# Autodesk Inventor assembly: HatpHexa
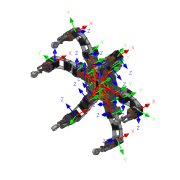
[picture p0: Inventor's stored thumbnail of the model, 180x180]
Saved by Autodesk Inventor 2019.4 (Build 234330000, 330)
## iProperties
Created: 2018-12-18
Part Number: HatpHexa
Material: 一般
Document SubType Name: Assembly
Designer: y6tada
Author: y6tada
## Documents named in this file (5)
- C:\Workspace\HaptHexa\Hardware\Inventor\HatpHexa.iam
- C:\Workspace\HaptHexa\Hardware\Inventor\Thorax\_Thorax.iam
- C:\Workspace\HaptHexa\Hardware\Inventor\Coxa\_Coxa.iam
- C:\Workspace\HaptHexa\Hardware\Inventor\Femur\_Femur.iam
- C:\Workspace\HaptHexa\Hardware\Inventor\Tibia\_Tibia.iam
## Components (19 placed, 4 different names)
1. _Thorax:1 [sub-assembly] — メイト:2, 角度:1, メイト:11, メイト:12, メイト:17, メイト:18, 角度:2, 角度:3, 角度:5, 角度:6, 角度:7, メイト:1, メイト:34, メイト:35, メイト:36, メイト:37, メイト:38, メイト:39
2. _Coxa:1 [sub-assembly] — メイト:1, 角度:1, メイト:2, メイト:44, メイト:45, 角度:8
3. _Femur:1 [sub-assembly] — メイト:44, メイト:45, メイト:46, メイト:47, 角度:8, 角度:9
4. _Tibia:1 [sub-assembly] — メイト:46, メイト:47, 角度:9
5. _Coxa:2 [sub-assembly] — メイト:11, メイト:12, 角度:2, メイト:48, メイト:49, 角度:10
6. _Femur:2 [sub-assembly] — メイト:48, メイト:49, メイト:50, メイト:51, 角度:10, 角度:11
7. _Tibia:2 [sub-assembly] — メイト:50, メイト:51, 角度:11
8. _Coxa:3 [sub-assembly] — メイト:17, メイト:18, 角度:3, メイト:52, メイト:53, 角度:12
9. _Femur:3 [sub-assembly] — メイト:52, メイト:53, メイト:54, メイト:55, 角度:12, 角度:13
10. _Tibia:3 [sub-assembly] — メイト:54, メイト:55, 角度:13
11. _Coxa:4 [sub-assembly] — メイト:36, メイト:39, メイト:56, メイト:57, 角度:5, 角度:14
12. _Femur:4 [sub-assembly] — メイト:56, メイト:57, メイト:58, メイト:59, 角度:14, 角度:15
13. _Tibia:4 [sub-assembly] — メイト:58, メイト:59, 角度:15
14. _Coxa:5 [sub-assembly] — メイト:35, メイト:37, 角度:6, メイト:60, メイト:61, 角度:16
15. _Femur:5 [sub-assembly] — メイト:60, メイト:61, メイト:62, メイト:63, 角度:16, 角度:17
16. _Tibia:5 [sub-assembly] — メイト:62, メイト:63, 角度:17
17. _Coxa:6 [sub-assembly] — メイト:34, メイト:38, メイト:40, メイト:41, 角度:7, 角度:18
18. _Femur:6 [sub-assembly] — メイト:40, メイト:41, メイト:42, メイト:43, 角度:18, 角度:19
19. _Tibia:6 [sub-assembly] — メイト:42, メイト:43, 角度:19
## Relationships (54: Mate 36, Angle 18)
- 角度:1 [Angle] (30 deg): _Thorax:1 ↔ _Coxa:1
- 角度:2 [Angle] (0 deg): _Thorax:1 ↔ _Coxa:2
- 角度:3 [Angle] (30 deg): _Thorax:1 ↔ _Coxa:3
- 角度:5 [Angle] (30 deg): _Thorax:1 ↔ _Coxa:4
- 角度:6 [Angle] (0 deg): _Thorax:1 ↔ _Coxa:5
- 角度:7 [Angle] (30 deg): _Thorax:1 ↔ _Coxa:6
- メイト:1 [Mate]: _Thorax:1 ↔ _Coxa:1
- メイト:2 [Mate]: _Thorax:1 ↔ _Coxa:1
- メイト:11 [Mate]: _Thorax:1 ↔ _Coxa:2
- メイト:12 [Mate]: _Thorax:1 ↔ _Coxa:2
- メイト:17 [Mate]: _Thorax:1 ↔ _Coxa:3
- メイト:18 [Mate]: _Thorax:1 ↔ _Coxa:3
- メイト:34 [Mate]: _Thorax:1 ↔ _Coxa:6
- メイト:35 [Mate]: _Thorax:1 ↔ _Coxa:5
- メイト:36 [Mate]: _Thorax:1 ↔ _Coxa:4
- メイト:37 [Mate]: _Thorax:1 ↔ _Coxa:5
- メイト:38 [Mate]: _Thorax:1 ↔ _Coxa:6
- メイト:39 [Mate]: _Thorax:1 ↔ _Coxa:4
- メイト:40 [Mate]: _Coxa:6 ↔ _Femur:6
- メイト:41 [Mate]: _Coxa:6 ↔ _Femur:6
- メイト:42 [Mate]: _Femur:6 ↔ _Tibia:6
- メイト:43 [Mate]: _Femur:6 ↔ _Tibia:6
- メイト:44 [Mate]: _Coxa:1 ↔ _Femur:1
- メイト:45 [Mate]: _Coxa:1 ↔ _Femur:1
- メイト:46 [Mate]: _Femur:1 ↔ _Tibia:1
- メイト:47 [Mate]: _Femur:1 ↔ _Tibia:1
- メイト:48 [Mate]: _Coxa:2 ↔ _Femur:2
- メイト:49 [Mate]: _Coxa:2 ↔ _Femur:2
- メイト:50 [Mate]: _Femur:2 ↔ _Tibia:2
- メイト:51 [Mate]: _Femur:2 ↔ _Tibia:2
- メイト:52 [Mate]: _Coxa:3 ↔ _Femur:3
- メイト:53 [Mate]: _Coxa:3 ↔ _Femur:3
- メイト:54 [Mate]: _Femur:3 ↔ _Tibia:3
- メイト:55 [Mate]: _Femur:3 ↔ _Tibia:3
- メイト:56 [Mate]: _Coxa:4 ↔ _Femur:4
- メイト:57 [Mate]: _Coxa:4 ↔ _Femur:4
- メイト:58 [Mate]: _Femur:4 ↔ _Tibia:4
- メイト:59 [Mate]: _Femur:4 ↔ _Tibia:4
- メイト:60 [Mate]: _Coxa:5 ↔ _Femur:5
- メイト:61 [Mate]: _Coxa:5 ↔ _Femur:5
- メイト:62 [Mate]: _Femur:5 ↔ _Tibia:5
- メイト:63 [Mate]: _Femur:5 ↔ _Tibia:5
- 角度:8 [Angle] (-10 deg): _Coxa:1 ↔ _Femur:1
- 角度:9 [Angle] (-80 deg): _Femur:1 ↔ _Tibia:1
- 角度:10 [Angle] (10 deg): _Coxa:2 ↔ _Femur:2
- 角度:11 [Angle] (80 deg): _Femur:2 ↔ _Tibia:2
- 角度:12 [Angle] (10 deg): _Coxa:3 ↔ _Femur:3
- 角度:13 [Angle] (80 deg): _Femur:3 ↔ _Tibia:3
- 角度:14 [Angle] (10 deg): _Coxa:4 ↔ _Femur:4
- 角度:15 [Angle] (80 deg): _Femur:4 ↔ _Tibia:4
- 角度:16 [Angle] (10 deg): _Coxa:5 ↔ _Femur:5
- 角度:17 [Angle] (-80 deg): _Femur:5 ↔ _Tibia:5
- 角度:18 [Angle] (-10 deg): _Coxa:6 ↔ _Femur:6
- 角度:19 [Angle] (-80 deg): _Femur:6 ↔ _Tibia:6
## Named parameters: femur_angle = 10 deg, tibia_angle = 80 deg
